# Autodesk Inventor assembly: Battery_Module
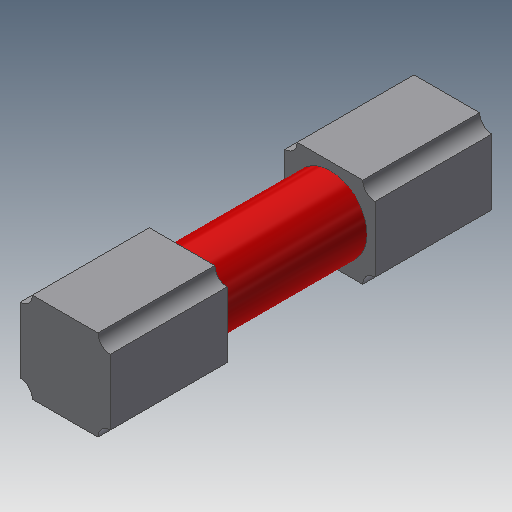
[picture p0: Inventor's stored thumbnail of the model, 512x512]
Saved by Autodesk Inventor 2018 (Build 220112000, 112)
## iProperties
Created: 2019-08-31
Part Number: Battery_Module
Document SubType Name: Assembly
Designer: Clevo
Author: Clevo
## Documents named in this file (3)
- E:\Hardware_Accelerated_Robot\Hardware\Battery\Battery_Module.iam
- E:\Hardware_Accelerated_Robot\Hardware\Battery\purecells.ipt
- E:\Hardware_Accelerated_Robot\Hardware\Battery\VRUZEND_Caps.ipt
## Components (3 placed, 2 different names)
1. purecells:1 — Mate:1, Mate:2, Mate:3, Mate:4
2. VRUZEND_Caps:1 — Mate:1, Mate:4, Flush:1, Angle:1
3. VRUZEND_Caps:2 — Mate:2, Mate:3, Flush:1
## Relationships (6: Mate 4, Flush 1, Angle 1)
- Mate:1: purecells:1 ↔ VRUZEND_Caps:1
- Mate:2: purecells:1 ↔ VRUZEND_Caps:2
- Mate:3: purecells:1 ↔ VRUZEND_Caps:2
- Mate:4: purecells:1 ↔ VRUZEND_Caps:1
- Flush:1: VRUZEND_Caps:1 ↔ VRUZEND_Caps:2
- Angle:1 (0 deg): VRUZEND_Caps:1
